# Autodesk Inventor assembly: lw_6_1_сборка_2
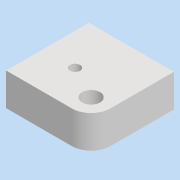
[picture p0: Inventor's stored thumbnail of the model, 180x180]
Saved by Autodesk Inventor 2022 (Build 260153000, 153)
## iProperties
Created: 2021-05-18
Part Number: lw_6_1_сборка_2
Document SubType Name: Assembly
Designer: Kurbatova
Author: Kurbatova
## Documents named in this file (3)
- C:\Users\Kurbatova\source\LW2021\LW_SAPR\лаб_6\lw_6_1_сборка_2.iam
- C:\Users\Kurbatova\source\LW2021\LW_SAPR\лаб_6\lw_6_part1.ipt
- C:\Users\Kurbatova\source\LW2021\LW_SAPR\лаб_6\lw_6_part2.ipt
## Components (2 placed, 2 different names)
1. lw_6_part1:1 — Заподлицо:1, Совмещение:1, Заподлицо:2
2. lw_6_part2:1 — Заподлицо:1, Совмещение:1, Заподлицо:2
## Relationships (3: Flush 2, Mate 1)
- Заподлицо:1 [Flush]: lw_6_part1:1 ↔ lw_6_part2:1
- Совмещение:1 [Mate]: lw_6_part1:1 ↔ lw_6_part2:1
- Заподлицо:2 [Flush]: lw_6_part1:1 ↔ lw_6_part2:1
